# Autodesk Inventor assembly: nc_nhk19
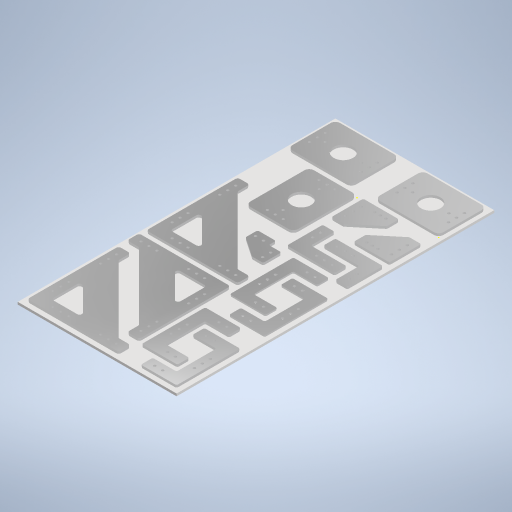
[picture p0: Inventor's stored thumbnail of the model, 512x512]
Saved by Autodesk Inventor 2023 (Build 270158000, 158)
## iProperties
Created: 2022-04-27
Part Number: nc_nhk19
Document SubType Name: Assembly
Designer: yuta
Author: yuta
## Documents named in this file (8)
- C:\Users\yuta\Documents\NHK\nc_nhk19.iam
- C:\Users\yuta\Documents\NHK\NC.port.ipt
- C:\Users\yuta\Documents\NHK\射出_固定2.ipt
- C:\Users\yuta\Documents\NHK\射出_固定1.ipt
- C:\Users\yuta\Documents\NHK\射出_固定6.ipt
- C:\Users\yuta\Documents\NHK\射出_エンコーダー固定.ipt
- C:\Users\yuta\Documents\NHK\射出_固定3.ipt
- C:\Users\yuta\Documents\NHK\射出_固定4.ipt
## Components (16 placed, 7 different names)
1. NC.port:1 — メイト:1, フラッシュ:1, フラッシュ:2, メイト:2, メイト:4, フラッシュ:3, メイト:6, フラッシュ:4, フラッシュ:5, メイト:7, フラッシュ:6, メイト:15, メイト:17, フラッシュ:7, メイト:20, フラッシュ:8, フラッシュ:9, メイト:21, フラッシュ:10, フラッシュ:11, メイト:22, フラッシュ:12, メイト:24, メイト:27, フラッシュ:13, メイト:29
2. 射出_固定2:1 — メイト:1, フラッシュ:1, フラッシュ:2, メイト:3
3. 射出_固定2:2 — メイト:2, メイト:3, メイト:5
4. 射出_固定2:3 — メイト:4, フラッシュ:3, メイト:5
5. 射出_固定1:1 — メイト:6, フラッシュ:4, フラッシュ:5, メイト:8, メイト:9
6. 射出_固定1:2 — メイト:7, メイト:8, メイト:9, メイト:14
7. 射出_固定1:3 — メイト:14, フラッシュ:6
8. 射出_固定1:4 — メイト:16, メイト:30
9. 射出_固定6:1 — メイト:15, メイト:16, メイト:18, メイト:19
10. 射出_固定6:2 — メイト:17, フラッシュ:7, メイト:18, メイト:19, メイト:28
11. 射出_エンコーダー固定:1 — メイト:20, フラッシュ:8, フラッシュ:9, メイト:23
12. 射出_エンコーダー固定:3 — メイト:21, フラッシュ:10, フラッシュ:11, メイト:26
13. 射出_エンコーダー固定:4 — メイト:22, メイト:23, フラッシュ:12, メイト:25, メイト:31
14. 射出_固定3:1 — メイト:27, メイト:28, フラッシュ:13
15. 射出_固定3:2 — メイト:24, メイト:25, メイト:26
16. 射出_固定4:1 — メイト:29, メイト:30, メイト:31
## Relationships (42: Mate 29, Flush 13)
- メイト:1 [Mate]: NC.port:1 ↔ 射出_固定2:1
- フラッシュ:1 [Flush] (6 mm): NC.port:1 ↔ 射出_固定2:1
- フラッシュ:2 [Flush] (6 mm): NC.port:1 ↔ 射出_固定2:1
- メイト:2 [Mate]: NC.port:1 ↔ 射出_固定2:2
- メイト:3 [Mate] (12 mm): 射出_固定2:1 ↔ 射出_固定2:2
- メイト:4 [Mate]: NC.port:1 ↔ 射出_固定2:3
- フラッシュ:3 [Flush] (6 mm): NC.port:1 ↔ 射出_固定2:3
- メイト:5 [Mate] (8 mm): 射出_固定2:2 ↔ 射出_固定2:3
- メイト:6 [Mate]: NC.port:1 ↔ 射出_固定1:1
- フラッシュ:4 [Flush] (6 mm): NC.port:1 ↔ 射出_固定1:1
- フラッシュ:5 [Flush] (6 mm): NC.port:1 ↔ 射出_固定1:1
- メイト:7 [Mate]: NC.port:1 ↔ 射出_固定1:2
- メイト:8 [Mate] (7 mm): 射出_固定1:1 ↔ 射出_固定1:2
- メイト:9 [Mate] (8 mm): 射出_固定1:1 ↔ 射出_固定1:2
- [Mate] (7 mm): 射出_固定1:3 ↔ 射出_固定1:4
- [Mate] (8 mm): 射出_固定1:3 ↔ 射出_固定1:4
- メイト:14 [Mate] (8 mm): 射出_固定1:2 ↔ 射出_固定1:3
- フラッシュ:6 [Flush] (6 mm): NC.port:1 ↔ 射出_固定1:3
- メイト:15 [Mate]: NC.port:1 ↔ 射出_固定6:1
- メイト:16 [Mate] (8 mm): 射出_固定1:4 ↔ 射出_固定6:1
- メイト:17 [Mate]: NC.port:1 ↔ 射出_固定6:2
- フラッシュ:7 [Flush] (6 mm): NC.port:1 ↔ 射出_固定6:2
- メイト:18 [Mate] (8 mm): 射出_固定6:1 ↔ 射出_固定6:2
- メイト:19 [Mate] (8 mm): 射出_固定6:1 ↔ 射出_固定6:2
- メイト:20 [Mate]: NC.port:1 ↔ 射出_エンコーダー固定:1
- フラッシュ:8 [Flush] (5 mm): NC.port:1 ↔ 射出_エンコーダー固定:1
- フラッシュ:9 [Flush] (5 mm): NC.port:1 ↔ 射出_エンコーダー固定:1
- メイト:21 [Mate]: NC.port:1 ↔ 射出_エンコーダー固定:3
- フラッシュ:10 [Flush] (5 mm): NC.port:1 ↔ 射出_エンコーダー固定:3
- フラッシュ:11 [Flush] (5 mm): NC.port:1 ↔ 射出_エンコーダー固定:3
- メイト:22 [Mate]: NC.port:1 ↔ 射出_エンコーダー固定:4
- メイト:23 [Mate] (8 mm): 射出_エンコーダー固定:1 ↔ 射出_エンコーダー固定:4
- フラッシュ:12 [Flush] (40 mm): NC.port:1 ↔ 射出_エンコーダー固定:4
- メイト:24 [Mate]: NC.port:1 ↔ 射出_固定3:2
- メイト:25 [Mate] (8 mm): 射出_エンコーダー固定:4 ↔ 射出_固定3:2
- メイト:26 [Mate] (8 mm): 射出_エンコーダー固定:3 ↔ 射出_固定3:2
- メイト:27 [Mate]: NC.port:1 ↔ 射出_固定3:1
- メイト:28 [Mate] (8 mm): 射出_固定6:2 ↔ 射出_固定3:1
- フラッシュ:13 [Flush] (6 mm): NC.port:1 ↔ 射出_固定3:1
- メイト:29 [Mate]: NC.port:1 ↔ 射出_固定4:1
- メイト:30 [Mate] (12 mm): 射出_固定1:4 ↔ 射出_固定4:1
- メイト:31 [Mate] (21 mm): 射出_エンコーダー固定:4 ↔ 射出_固定4:1
## Named parameters: d14_d12 = 7 mm, d15_d13 = 8 mm
